# Autodesk Inventor assembly: Robot
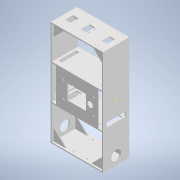
[picture p0: Inventor's stored thumbnail of the model, 180x180]
Saved by Autodesk Inventor 2020 (Build 240168000, 168)
## iProperties
Created: 2020-01-31
Part Number: Robot
Document SubType Name: Assembly
Designer: jelte
Author: jelte
## Documents named in this file (8)
- E:\GIP\EA\3D Tekeningen\Versie 2\Robot.iam
- E:\GIP\EA\3D Tekeningen\Versie 2\Muur.ipt
- E:\GIP\EA\3D Tekeningen\Versie 2\Level1 (Motoren).ipt
- E:\GIP\EA\3D Tekeningen\Versie 2\Level2 (Arduino).ipt
- E:\GIP\EA\3D Tekeningen\Versie 2\Level3 (Voeding).ipt
- E:\GIP\EA\3D Tekeningen\Versie 2\Level4 (Sensor + Schakelaars).ipt
- E:\GIP\EA\3D Tekeningen\Versie 2\Level2-3 (GLCD).ipt
- E:\GIP\EA\3D Tekeningen\Versie 2\Support Piece.ipt
## Components (15 placed, 7 different names)
1. Muur:1 — Rigid:1, Rigid:5, Rigid:6, Rigid:7, Rigid:16, Rigid:17, Rigid:20, Rigid:21
2. Level1 (Motoren):1 — Rigid:1
3. Level2 (Arduino):1 — Rigid:5
4. Level3 (Voeding):1 — Rigid:6, Rigid:15
5. Level4 (Sensor + Schakelaars):1 — Rigid:7, Rigid:8
6. Muur:2 — Rigid:8, Rigid:18, Rigid:19, Rigid:22, Rigid:23
7. Level2-3 (GLCD):1 — Rigid:15
8. Support Piece:1 — Rigid:16
9. Support Piece:2 — Rigid:17
10. Support Piece:3 — Rigid:19
11. Support Piece:4 — Rigid:18
12. Support Piece:5 — Rigid:20
13. Support Piece:6 — Rigid:21
14. Support Piece:7 — Rigid:23
15. Support Piece:8 — Rigid:22
## Relationships (14: WeldJoint 14)
- Rigid:1 [WeldJoint]: Muur:1 ↔ Level1 (Motoren):1
- Rigid:5 [WeldJoint]: Muur:1 ↔ Level2 (Arduino):1
- Rigid:6 [WeldJoint]: Muur:1 ↔ Level3 (Voeding):1
- Rigid:7 [WeldJoint]: Muur:1 ↔ Level4 (Sensor + Schakelaars):1
- Rigid:8 [WeldJoint]: Level4 (Sensor + Schakelaars):1 ↔ Muur:2
- Rigid:15 [WeldJoint]: Level3 (Voeding):1 ↔ Level2-3 (GLCD):1
- Rigid:16 [WeldJoint]: Muur:1 ↔ Support Piece:1
- Rigid:17 [WeldJoint]: Muur:1 ↔ Support Piece:2
- Rigid:18 [WeldJoint]: Muur:2 ↔ Support Piece:4
- Rigid:19 [WeldJoint]: Muur:2 ↔ Support Piece:3
- Rigid:20 [WeldJoint]: Muur:1 ↔ Support Piece:5
- Rigid:21 [WeldJoint]: Muur:1 ↔ Support Piece:6
- Rigid:22 [WeldJoint]: Muur:2 ↔ Support Piece:8
- Rigid:23 [WeldJoint]: Muur:2 ↔ Support Piece:7
